# Autodesk Inventor assembly: LIA0001-SHELF
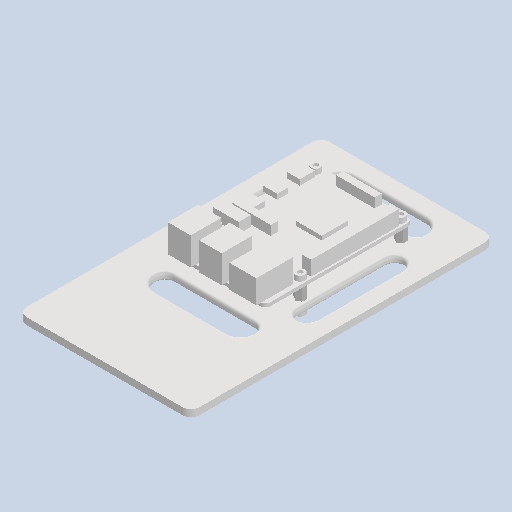
[picture p0: Inventor's stored thumbnail of the model, 512x512]
Saved by Autodesk Inventor 2023 (Build 270158000, 158)
## iProperties
Created: 2023-03-17
Part Number: LIA0001-SHELF
Document SubType Name: Assembly
Designer: Louis
Author: Louis
## Documents named in this file (7)
- D:\Louis\Documents\Inventor\Interferometry\LIA0001-SHELF.iam
- D:\Louis\Documents\Inventor\Interferometry\LI0003-COMPONENT SHELF.ipt
- D:\Louis\Documents\Inventor\Interferometry\PI 4 B SPACE MODEL.ipt
- D:\Louis\Documents\Inventor\Interferometry\ACCU HHTPS-M3-5-8-S-Z.ipt
- D:\Louis\Documents\Inventor\Interferometry\M3 WASHER.ipt
- D:\Louis\Documents\Inventor\Interferometry\M3 X 6.ipt
- D:\Louis\Documents\Inventor\Interferometry\LI0015-PI B DIE.ipt
## Components (19 placed, 6 different names)
1. LI0003-COMPONENT SHELF:1 — Mate:1, Mate:2, Mate:3, Insert:2, Insert:3, Insert:4, Insert:7, Insert:12, Insert:13, Insert:14, Insert:15
2. PI 4 B SPACE MODEL:1 — Insert:8, Insert:9, Insert:10, Insert:11, Insert:16, Insert:17, Insert:18, Insert:19, Mate:4, Flush:1, Flush:2
3. ACCU HHTPS-M3-5-8-S-Z:1 — Insert:7, Insert:10
4. ACCU HHTPS-M3-5-8-S-Z:2 — Insert:2, Insert:8
5. ACCU HHTPS-M3-5-8-S-Z:3 — Insert:4, Insert:11
6. ACCU HHTPS-M3-5-8-S-Z:4 — Insert:3, Insert:9
7. M3 WASHER:1 — Insert:13, Insert:22
8. M3 WASHER:2 — Insert:14, Insert:20
9. M3 WASHER:4 — Insert:15, Insert:23
10. M3 WASHER:8 — Insert:12, Insert:21
11. M3 X 6:1 — Insert:22
12. M3 X 6:2 — Insert:23
13. M3 X 6:3 — Insert:21
14. M3 X 6:4 — Insert:19
15. M3 X 6:5 — Insert:20
16. M3 X 6:6 — Insert:17
17. M3 X 6:7 — Insert:16
18. M3 X 6:8 — Insert:18
19. LI0015-PI B DIE:1 — Mate:4, Flush:1, Flush:2
## Relationships (26: Insert 20, Mate 4, Flush 2)
- Mate:1: LI0003-COMPONENT SHELF:1
- Mate:2: LI0003-COMPONENT SHELF:1
- Mate:3: LI0003-COMPONENT SHELF:1
- Insert:2: LI0003-COMPONENT SHELF:1 ↔ ACCU HHTPS-M3-5-8-S-Z:2
- Insert:3: LI0003-COMPONENT SHELF:1 ↔ ACCU HHTPS-M3-5-8-S-Z:4
- Insert:4: LI0003-COMPONENT SHELF:1 ↔ ACCU HHTPS-M3-5-8-S-Z:3
- Insert:7: LI0003-COMPONENT SHELF:1 ↔ ACCU HHTPS-M3-5-8-S-Z:1
- Insert:8: PI 4 B SPACE MODEL:1 ↔ ACCU HHTPS-M3-5-8-S-Z:2
- Insert:9: PI 4 B SPACE MODEL:1 ↔ ACCU HHTPS-M3-5-8-S-Z:4
- Insert:10: PI 4 B SPACE MODEL:1 ↔ ACCU HHTPS-M3-5-8-S-Z:1
- Insert:11: PI 4 B SPACE MODEL:1 ↔ ACCU HHTPS-M3-5-8-S-Z:3
- Insert:12: LI0003-COMPONENT SHELF:1 ↔ M3 WASHER:8
- Insert:13: LI0003-COMPONENT SHELF:1 ↔ M3 WASHER:1
- Insert:14: LI0003-COMPONENT SHELF:1 ↔ M3 WASHER:2
- Insert:15: LI0003-COMPONENT SHELF:1 ↔ M3 WASHER:4
- Insert:16: PI 4 B SPACE MODEL:1 ↔ M3 X 6:7
- Insert:17: PI 4 B SPACE MODEL:1 ↔ M3 X 6:6
- Insert:18: PI 4 B SPACE MODEL:1 ↔ M3 X 6:8
- Insert:19: PI 4 B SPACE MODEL:1 ↔ M3 X 6:4
- Insert:20: M3 WASHER:2 ↔ M3 X 6:5
- Insert:21: M3 WASHER:8 ↔ M3 X 6:3
- Insert:22: M3 WASHER:1 ↔ M3 X 6:1
- Insert:23: M3 WASHER:4 ↔ M3 X 6:2
- Mate:4: PI 4 B SPACE MODEL:1 ↔ LI0015-PI B DIE:1
- Flush:1: PI 4 B SPACE MODEL:1 ↔ LI0015-PI B DIE:1
- Flush:2: PI 4 B SPACE MODEL:1 ↔ LI0015-PI B DIE:1
